# Autodesk Inventor assembly: wheel shaft
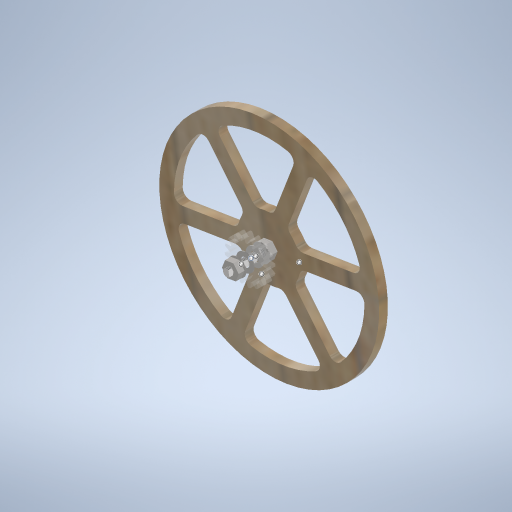
[picture p0: Inventor's stored thumbnail of the model, 512x512]
Saved by Autodesk Inventor 2023 (Build 270158000, 158)
## iProperties
Created: 2023-06-05
Part Number: wheel shaft
Document SubType Name: Assembly
Designer: Ronan
Author: Ronan
## Documents named in this file (6)
- D:\Libraries\Documents\2023-FYP\Inventor\wheel shaft.iam
- D:\Libraries\Documents\2023-FYP\Inventor\Assembly\Design Accelerator\Spur Gear22.ipt
- D:\Libraries\Documents\2023-FYP\Inventor\m5-screw-cut.ipt
- D:\Libraries\Documents\2023-FYP\Inventor\Wheel.iam
- D:\Libraries\Documents\2023-FYP\Inventor\M5-nut-4mm.ipt
- D:\Libraries\Documents\2023-FYP\Inventor\M5-washer.ipt
## Components (9 placed, 5 different names)
1. Spur Gear2:1 — Mate:10, Cylindrical:4, Mate:11, Mate:12
2. m5-screw-cut:1 — Cylindrical:4, Cylindrical:5, Cylindrical:6
3. Wheel:1 [sub-assembly]
4. M5-nut-4mm:1 — Flush:2
5. M5-washer:1
6. M5-washer:2 — Mate:10
7. M5-nut-4mm:2 — Flush:2
8. M5-washer:3 — Mate:11, Cylindrical:6
9. M5-washer:4 — Mate:12, Cylindrical:5
## Relationships (20: Mate 12, CylindricalJoint 6, Flush 2)
- [Mate]: Spur Gear2:1 ↔ m5-screw-cut:1
- [Mate]: m5-screw-cut:1 ↔ Wheel:1
- [Mate]: m5-screw-cut:1 ↔ Wheel:1
- [Mate]: m5-screw-cut:1 ↔ Wheel:1
- [Flush]: Wheel:1 ↔ M5-nut-4mm:1
- [Mate]: m5-screw-cut:1 ↔ M5-nut-4mm:1
- [Mate] (0.01 mm): Wheel:1 ↔ M5-nut-4mm:1
- [CylindricalJoint]: m5-screw-cut:1 ↔ M5-washer:1
- [Mate] (0.01 mm): M5-nut-4mm:1 ↔ M5-washer:1
- [Mate]: Spur Gear2:1 ↔ m5-screw-cut:1
- [CylindricalJoint]: m5-screw-cut:1 ↔ M5-washer:2
- [CylindricalJoint]: m5-screw-cut:1 ↔ M5-nut-4mm:2
- [Mate] (0.5 mm): M5-washer:2 ↔ M5-nut-4mm:2
- Mate:10 (5.5 mm): Spur Gear2:1 ↔ M5-washer:2
- Cylindrical:4: Spur Gear2:1 ↔ m5-screw-cut:1
- Flush:2: M5-nut-4mm:1 ↔ M5-nut-4mm:2
- Mate:11: Spur Gear2:1 ↔ M5-washer:3
- Mate:12: Spur Gear2:1 ↔ M5-washer:4
- Cylindrical:5: m5-screw-cut:1 ↔ M5-washer:4
- Cylindrical:6: m5-screw-cut:1 ↔ M5-washer:3
